# Autodesk Inventor assembly: Vertical Strut
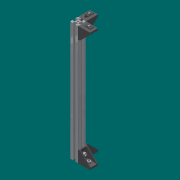
[picture p0: Inventor's stored thumbnail of the model, 180x180]
Saved by Autodesk Inventor 2016 SP1 (Build 200210100, 210)
## iProperties
Created: 2015-06-02
Part Number: Vertical Strut
Document SubType Name: Assembly
Designer: Sawaiz Syed
Author: Sawaiz Syed
## Documents named in this file (3)
- C:\Users\Sawaiz\OneDrive\projects\modularRICH\testMount\frame\verticalStrut.iam
- C:\Users\Sawaiz\OneDrive\projects\modularRICH\testMount\frame\hfs5-2020OrthagonalBeamHeight.ipt
- C:\Users\Sawaiz\OneDrive\projects\modularRICH\testMount\frame\angleBracket.iam
## Components (5 placed, 2 different names)
1. hfs5-2020OrthagonalBeamHeight:1 — Flush:3, Flush:4, Flush:5, Flush:6, Flush:7, Flush:8, Mate:1, Mate:2, Mate:3, Mate:4
2. angleBracket:1 [sub-assembly] — Flush:1, Flush:6, Mate:2
3. angleBracket:2 [sub-assembly] — Flush:1, Flush:4, Flush:5, Mate:1
4. angleBracket:3 [sub-assembly] — Flush:2, Flush:8, Mate:3
5. angleBracket:4 [sub-assembly] — Flush:2, Flush:3, Flush:7, Mate:4
## Relationships (12: Flush 8, Mate 4)
- Flush:1: angleBracket:1 ↔ angleBracket:2
- Flush:2: angleBracket:3 ↔ angleBracket:4
- Flush:3: hfs5-2020OrthagonalBeamHeight:1 ↔ angleBracket:4
- Flush:4: hfs5-2020OrthagonalBeamHeight:1 ↔ angleBracket:2
- Flush:5: hfs5-2020OrthagonalBeamHeight:1 ↔ angleBracket:2
- Flush:6: hfs5-2020OrthagonalBeamHeight:1 ↔ angleBracket:1
- Flush:7: hfs5-2020OrthagonalBeamHeight:1 ↔ angleBracket:4
- Flush:8: hfs5-2020OrthagonalBeamHeight:1 ↔ angleBracket:3
- Mate:1: hfs5-2020OrthagonalBeamHeight:1 ↔ angleBracket:2
- Mate:2: hfs5-2020OrthagonalBeamHeight:1 ↔ angleBracket:1
- Mate:3: hfs5-2020OrthagonalBeamHeight:1 ↔ angleBracket:3
- Mate:4: hfs5-2020OrthagonalBeamHeight:1 ↔ angleBracket:4
